# Autodesk Inventor assembly: EL2-500
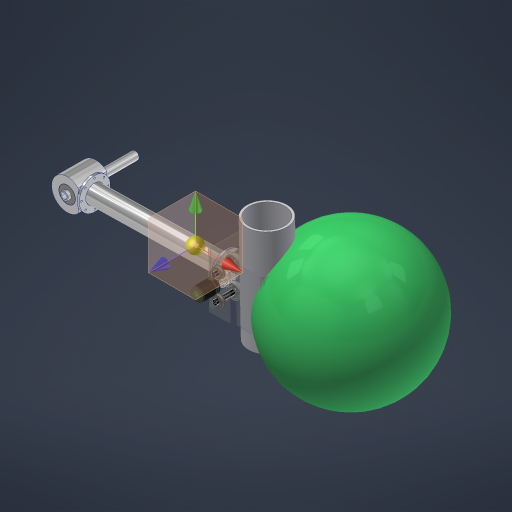
[picture p0: Inventor's stored thumbnail of the model, 512x512]
Saved by Autodesk Inventor 2023.4 (Build 274418000, 418)
## iProperties
Created: 2025-01-18
Part Number: EL2-500
Document SubType Name: Assembly
Designer: brand
Mass: 3982.19 g
Surface Area: 12146.7 cm^2
Volume: 36904 cm^3
Density: 0.107907 g/cm^3
Author: brand
## Documents named in this file (4)
- C:\Users\brand\OneDrive\Documents\GitHub\robotics 23\2025-ReefScape---CAD\Elevator\EL2\EL2-500.iam
- C:\Users\brand\OneDrive\Documents\GitHub\robotics 23\2025-ReefScape---CAD\Gripper\GP3\GP3-100.iam
- C:\Users\brand\OneDrive\Documents\GitHub\robotics 23\2025-ReefScape---CAD\Elevator\EL2\EL2-A-100.iam
- C:\Users\brand\OneDrive\Documents\GitHub\robotics 23\2025-ReefScape---CAD\Field Items\Game Pieces\GE-25501.ipt
## Components (3 placed, 3 different names)
1. EL2-A-100:1 [sub-assembly] — Insert:1, Insert:2
2. GP3-100:1 [sub-assembly] — Insert:1, Insert:2
3. GE-25501:1
## Relationships (2: Insert 2)
- Insert:1: EL2-A-100:1 ↔ GP3-100:1
- Insert:2: EL2-A-100:1 ↔ GP3-100:1
